# Autodesk Inventor assembly: Assembly1
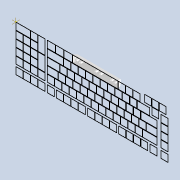
[picture p0: Inventor's stored thumbnail of the model, 180x180]
Saved by Autodesk Inventor 2021 (Build 250183000, 183)
## iProperties
Created: 2021-12-04
Part Number: Assembly1
Document SubType Name: Assembly
Designer: Matthew Flooks
Author: Matthew Flooks
## Documents named in this file (3)
- C:\Users\Matthew Flooks\Documents\GitHub\QEX103-PCB\3D Model\Assembly1.iam
- C:\Users\Matthew Flooks\Documents\GitHub\QEX103-PCB\3D Model\Layout.ipt
- C:\Users\Matthew Flooks\Documents\GitHub\QEX103-PCB\3D Model\KeyCaps\Space.ipt
## Components (2 placed, 2 different names)
1. Layout:1 — Mate:1, Mate:2, Mate:3, Mate:4
2. Space:1 — Mate:3, Mate:4
## Relationships (4: Mate 4)
- Mate:1: Layout:1
- Mate:2: Layout:1
- Mate:3: Layout:1 ↔ Space:1
- Mate:4: Layout:1 ↔ Space:1
